# Autodesk Inventor assembly: Assembly1
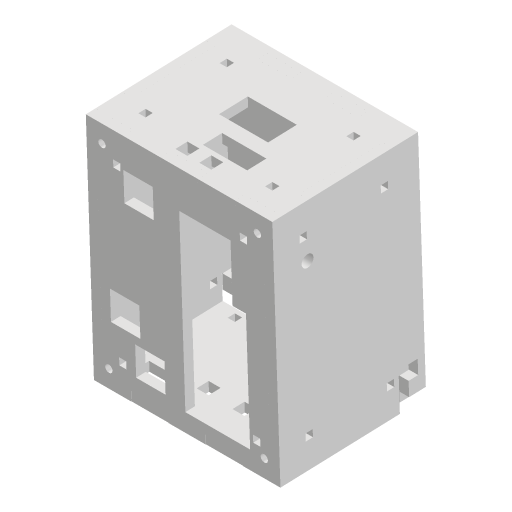
[picture p0: Inventor's stored thumbnail of the model, 512x512]
Saved by Autodesk Inventor 2023.3 (Build 273359000, 359)
## iProperties
Created: 2024-06-25
Part Number: Assembly1
Document SubType Name: Assembly
Designer: David Zindović
Author: David Zindović
## Documents named in this file (7)
- C:\Users\David Zindović\Desktop\Projekti\FE LMK\Poletna Sola\Ohisje\Assembly1.iam
- C:\Users\David Zindović\Desktop\Projekti\FE LMK\Poletna Sola\Ohisje\Bottom.ipt
- C:\Users\David Zindović\Desktop\Projekti\FE LMK\Poletna Sola\Ohisje\Side.ipt
- C:\Users\David Zindović\Desktop\Projekti\FE LMK\Poletna Sola\Ohisje\Back.ipt
- C:\Users\David Zindović\Desktop\Projekti\FE LMK\Poletna Sola\Ohisje\Front.ipt
- C:\Users\David Zindović\Desktop\Projekti\FE LMK\Poletna Sola\Ohisje\Top.ipt
- C:\Users\David Zindović\Desktop\Projekti\FE LMK\Poletna Sola\Ohisje\Side DRUGA STRAN.ipt
## Components (6 placed, 6 different names)
1. Bottom:1 — Flush:21, Mate:9, Flush:22
2. Side DRUGA STRAN:1
3. Side:2 — Flush:14, Flush:15, Flush:22, Flush:24, Flush:26, Flush:27
4. Back:1 — Flush:25, Flush:26, Flush:27
5. Front:1 — Flush:14, Flush:15, Flush:21, Mate:9, Flush:23
6. Top:1 — Flush:23, Flush:24, Flush:25
## Relationships (17: Flush 15, Mate 2)
- [Flush]: Side DRUGA STRAN:1 ↔ Front:1
- [Flush]: Bottom:1 ↔ Side DRUGA STRAN:1
- [Flush]: Side DRUGA STRAN:1 ↔ Front:1
- [Mate]: Side DRUGA STRAN:1 ↔ Front:1
- [Flush]: Side DRUGA STRAN:1 ↔ Front:1
- Flush:14: Side:2 ↔ Front:1
- Flush:15: Side:2 ↔ Front:1
- [Flush]: Side DRUGA STRAN:1 ↔ Top:1
- [Flush]: Side DRUGA STRAN:1 ↔ Top:1
- Flush:21: Bottom:1 ↔ Front:1
- Mate:9: Bottom:1 ↔ Front:1
- Flush:22: Bottom:1 ↔ Side:2
- Flush:23: Front:1 ↔ Top:1
- Flush:24: Side:2 ↔ Top:1
- Flush:25: Back:1 ↔ Top:1
- Flush:26: Side:2 ↔ Back:1
- Flush:27: Side:2 ↔ Back:1
